# Autodesk Inventor assembly: Assembly2
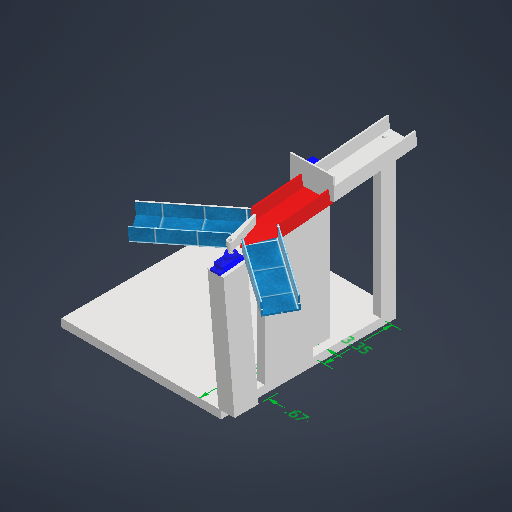
[picture p0: Inventor's stored thumbnail of the model, 512x512]
Saved by Autodesk Inventor 2026.2 (Build 302298000, 298)
## iProperties
Created: 2026-02-23
Part Number: Assembly2
Document SubType Name: Assembly
Designer: danda
Author: danda
## Documents named in this file (13)
- C:\Users\danda\OneDrive\Desktop\Basics Of Mecha\Project\sorting\Assembly2.iam
- C:\Users\danda\OneDrive\Desktop\Basics Of Mecha\Project\sorting\stand.ipt
- C:\Users\danda\OneDrive\Desktop\Basics Of Mecha\Project\sorting\stand2.ipt
- C:\Users\danda\OneDrive\Desktop\Basics Of Mecha\Project\sorting\inslide.ipt
- C:\Users\danda\OneDrive\Desktop\Basics Of Mecha\Project\sorting\base.ipt
- C:\Users\danda\OneDrive\Desktop\Basics Of Mecha\Project\sorting\Towerpro Micro Servo 9g\Towerpro Micro Servo 9g\Towerpro Micro Servo 9g.ipt
- C:\Users\danda\OneDrive\Desktop\Basics Of Mecha\Project\sorting\motorstand1.ipt
- C:\Users\danda\OneDrive\Desktop\Basics Of Mecha\Project\sorting\gate.ipt
- C:\Users\danda\OneDrive\Desktop\Basics Of Mecha\Project\sorting\middleslide.ipt
- C:\Users\danda\OneDrive\Desktop\Basics Of Mecha\Project\sorting\motorstand2.ipt
- C:\Users\danda\OneDrive\Desktop\Basics Of Mecha\Project\sorting\gate2.ipt
- C:\Users\danda\OneDrive\Desktop\Basics Of Mecha\Project\sorting\outslide.ipt
- C:\Users\danda\OneDrive\Desktop\Basics Of Mecha\Project\sorting\outslideleft.ipt
## Components (13 placed, 12 different names)
1. stand:1 — Mate:5, Flush:8, Flush:9, Mate:30, Mate:33, Flush:14, Mate:34
2. stand2:1 — Mate:4, Flush:1, Flush:7, Mate:17, Mate:18, Mate:30, Mate:31, Mate:32, Flush:13
3. inslide:1 — Flush:8, Mate:17, Mate:18, Mate:31, Mate:32, Flush:13
4. base:1 — Mate:3, Mate:4, Flush:1, Mate:5, Mate:9, Mate:14, Mate:15, Flush:7, Flush:12, Flush:15, Mate:39, Mate:40, Mate:41
5. Towerpro Micro Servo 9g:1 — Mate:11, Mate:12, Mate:13, Insert:1
6. motorstand1:1 — Mate:9, Mate:11, Mate:12, Mate:13, Flush:12, Flush:15
7. gate:1 — Insert:1
8. middleslide:1 — Flush:9, Mate:33, Flush:14, Mate:34, Flush:16, Mate:35, Mate:36, Mate:37, Flush:17, Mate:38
9. motorstand2:1 — Mate:21, Mate:22, Mate:23, Mate:39, Mate:40, Mate:41
10. Towerpro Micro Servo 9g:2 — Mate:21, Mate:22, Mate:23, Insert:2, Rotational:1
11. gate2:1 — Insert:2, Rotational:1
12. outslide:1 — Flush:16, Mate:35, Mate:36
13. outslideleft:1 — Mate:37, Flush:17, Mate:38
## Relationships (39: Mate 26, Flush 10, Insert 2, RevoluteJoint 1)
- Mate:3: base:1
- Mate:4: stand2:1 ↔ base:1
- Flush:1: stand2:1 ↔ base:1
- Mate:5: stand:1 ↔ base:1
- Mate:9: base:1 ↔ motorstand1:1
- Mate:11: Towerpro Micro Servo 9g:1 ↔ motorstand1:1
- Mate:12: Towerpro Micro Servo 9g:1 ↔ motorstand1:1
- Mate:13: Towerpro Micro Servo 9g:1 ↔ motorstand1:1
- Insert:1: Towerpro Micro Servo 9g:1 ↔ gate:1
- Mate:14: base:1
- Mate:15: base:1
- Flush:7: stand2:1 ↔ base:1
- Flush:8: stand:1 ↔ inslide:1
- Mate:17: stand2:1 ↔ inslide:1
- Mate:18: stand2:1 ↔ inslide:1
- Flush:9: stand:1 ↔ middleslide:1
- Mate:21: motorstand2:1 ↔ Towerpro Micro Servo 9g:2
- Mate:22: motorstand2:1 ↔ Towerpro Micro Servo 9g:2
- Mate:23: motorstand2:1 ↔ Towerpro Micro Servo 9g:2
- Insert:2: Towerpro Micro Servo 9g:2 ↔ gate2:1
- Flush:12 (119.38 mm): base:1 ↔ motorstand1:1
- Mate:30 (85 mm): stand:1 ↔ stand2:1
- Mate:31: stand2:1 ↔ inslide:1
- Mate:32: stand2:1 ↔ inslide:1
- Flush:13: stand2:1 ↔ inslide:1
- Mate:33: stand:1 ↔ middleslide:1
- Flush:14: stand:1 ↔ middleslide:1
- Mate:34: stand:1 ↔ middleslide:1
- Flush:15 (10.16 mm): base:1 ↔ motorstand1:1
- Flush:16: middleslide:1 ↔ outslide:1
- Mate:35: middleslide:1 ↔ outslide:1
- Mate:36: middleslide:1 ↔ outslide:1
- Mate:37: middleslide:1 ↔ outslideleft:1
- Flush:17: middleslide:1 ↔ outslideleft:1
- Mate:38: middleslide:1 ↔ outslideleft:1
- Rotational:1 [RevoluteJoint]: Towerpro Micro Servo 9g:2 ↔ gate2:1
- Mate:39: base:1 ↔ motorstand2:1
- Mate:40: base:1 ↔ motorstand2:1
- Mate:41 (17.018 mm): base:1 ↔ motorstand2:1
## Named parameters: Finish1_Area = 245.596, Finish2_Area = 72.4327
note: some values were not read from the file. Shown as the stored number, unit unknown: "Finish1_Area", "Finish2_Area".
